# Autodesk Inventor assembly: Assembly
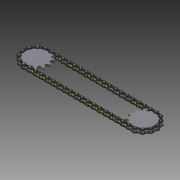
[picture p0: Inventor's stored thumbnail of the model, 180x180]
Saved by Autodesk Inventor 2014 (Build 180170000, 170)
## iProperties
Created: 2013-07-16
Part Number: Assembly
Document SubType Name: Assembly
Designer: Mill
Author: Mill
## Documents named in this file (4)
- C:\Users\Mill\Downloads\Chain\Assembly.iam
- C:\Users\Mill\Downloads\Chain\Master.ipt
- C:\Users\Mill\Downloads\Chain\ConnectingLinks.ipt
- C:\Users\Mill\Downloads\Chain\Roller Chain Sprocket11.ipt
## Components (53 placed, 3 different names)
1. Master:1 — Flush:1, Flush:2, Flush:3, Mate:1, Drive, Mate:6
2. Roller Chain Sprocket1:1 — Mate:4, Mate:5, Angle:3, Rotation:1
3. Roller Chain Sprocket1:2 — Mate:7, Mate:8, QUAY, Rotation:1
4. ConnectingLinks:1 — Mate:1, Angle:1, Mate:2
5. ConnectingLinks:2
6. ConnectingLinks:3
7. ConnectingLinks:4
8. ConnectingLinks:5
9. ConnectingLinks:6
10. ConnectingLinks:7
11. ConnectingLinks:8
12. ConnectingLinks:9
13. ConnectingLinks:10
14. ConnectingLinks:11
15. ConnectingLinks:12
16. ConnectingLinks:13
17. ConnectingLinks:14
18. ConnectingLinks:15
19. ConnectingLinks:16
20. ConnectingLinks:17
21. ConnectingLinks:18
22. ConnectingLinks:19
23. ConnectingLinks:20
24. ConnectingLinks:21
25. ConnectingLinks:22
26. ConnectingLinks:23
27. ConnectingLinks:24
28. ConnectingLinks:25
29. ConnectingLinks:26
30. ConnectingLinks:27
31. ConnectingLinks:28
32. ConnectingLinks:29
33. ConnectingLinks:30
34. ConnectingLinks:31
35. ConnectingLinks:32
36. ConnectingLinks:33
37. ConnectingLinks:34
38. ConnectingLinks:35
39. ConnectingLinks:36
40. ConnectingLinks:37
41. ConnectingLinks:38
42. ConnectingLinks:39
43. ConnectingLinks:40
44. ConnectingLinks:41
45. ConnectingLinks:42
46. ConnectingLinks:43
47. ConnectingLinks:44
48. ConnectingLinks:45
49. ConnectingLinks:46
50. ConnectingLinks:47
51. ConnectingLinks:48
52. ConnectingLinks:49
53. ConnectingLinks:50
## Component patterns: (50 elements, first: ConnectingLinks:1)
## Relationships (16: Mate 8, Angle 4, Flush 3, RelateRotation 1)
- Flush:1: Master:1
- Flush:2: Master:1
- Flush:3: Master:1
- Mate:1: Master:1 ↔ ConnectingLinks:1
- Angle:1 (0 deg): ConnectingLinks:1
- Mate:2: ConnectingLinks:1
- Drive [Mate] (234.95 mm): Master:1
- Mate:4: Roller Chain Sprocket1:1
- Mate:5: Roller Chain Sprocket1:1
- Mate:6: Master:1
- Angle:2 (0 deg)
- Mate:7: Roller Chain Sprocket1:2
- Mate:8: Roller Chain Sprocket1:2
- Angle:3 (0 deg): Roller Chain Sprocket1:1
- QUAY [Angle] (180 deg): Roller Chain Sprocket1:2
- Rotation:1 [RelateRotation] (1 ul): Roller Chain Sprocket1:1 ↔ Roller Chain Sprocket1:2
